# Autodesk Inventor assembly: complete
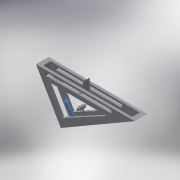
[picture p0: Inventor's stored thumbnail of the model, 180x180]
Saved by Autodesk Inventor 2019 (Build 230136000, 136)
## iProperties
Created: 2020-03-04
Part Number: complete
Document SubType Name: Assembly
Designer: HP
Author: HP
## Documents named in this file (4)
- C:\Users\HP\Desktop\manoj\complete.iam
- C:\Users\HP\Desktop\manoj\FINAL FRUSTATED.....iam
- C:\Users\HP\Desktop\manoj\ballholder1.iam
- C:\Users\HP\Desktop\manoj\pullyy.iam
## Components (3 placed, 3 different names)
1. FINAL FRUSTATED....:1 [sub-assembly] — Rigid:1, Mate:1
2. ballholder1:1 [sub-assembly] — Rigid:1
3. pullyy:1 [sub-assembly] — Mate:1
## Relationships (2: WeldJoint 1, Mate 1)
- Rigid:1 [WeldJoint]: FINAL FRUSTATED....:1 ↔ ballholder1:1
- Mate:1: FINAL FRUSTATED....:1 ↔ pullyy:1
